# Autodesk Inventor assembly: Ensamble_Amortiguador
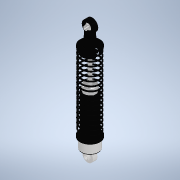
[picture p0: Inventor's stored thumbnail of the model, 180x180]
Saved by Autodesk Inventor 2020.2 (Build 242310000, 310)
## iProperties
Created: 2019-10-03
Part Number: Ensamble_Amortiguador
Document SubType Name: Assembly
Designer: axelj
Author: axelj
## Documents named in this file (11)
- C:\Users\axelj\OneDrive\Documentos\GitHub\autobot\robot_model\Ensamble_Amortiguador.iam
- C:\Users\axelj\OneDrive\Documentos\GitHub\autobot\robot_model\RCT-T005_Piston(Deposito_deAceite).ipt
- C:\Users\axelj\OneDrive\Documentos\GitHub\autobot\robot_model\RCT-T005_Embolo.ipt
- C:\Users\axelj\OneDrive\Documentos\GitHub\autobot\robot_model\RCT-T005_Elemento_externo.ipt
- C:\Users\axelj\OneDrive\Documentos\GitHub\autobot\robot_model\RCT-T005_Resorte.ipt
- C:\Users\axelj\OneDrive\Documentos\GitHub\autobot\robot_model\RCT-T005_Cubierta.ipt
- C:\Users\axelj\OneDrive\Documentos\GitHub\autobot\robot_model\RCT-T005_Conexion_superioript.ipt
- C:\Users\axelj\OneDrive\Documentos\GitHub\autobot\robot_model\RCT-T005_Pieza_Presion_resorte.ipt
- C:\Users\axelj\OneDrive\Documentos\GitHub\autobot\robot_model\RCT-T005_Conexion_inferior.ipt
- C:\Users\axelj\OneDrive\Documentos\GitHub\autobot\robot_model\RCT-H017_Bola_de_libertad_menor.ipt
- C:\Users\axelj\OneDrive\Documentos\GitHub\autobot\robot_model\RCT-H015_Bola_libertad_grande.ipt
## Components (10 placed, 10 different names)
1. RCT-T005_Piston(Deposito_deAceite):1 — Cilíndrica:1, Rígido:1, De rotación:1, De rotación:3
2. RCT-T005_Embolo:1 — Cilíndrica:1, De rotación:2
3. RCT-T005_Elemento_externo:1 — Rígido:1
4. RCT-T005_Resorte:1
5. RCT-T005_Cubierta:1 — De rotación:1
6. RCT-T005_Conexion_superioript:1 — De rotación:2, Rígido:2, De bola:1
7. RCT-T005_Pieza_Presion_resorte:1 — Rígido:2
8. RCT-T005_Conexion_inferior:1 — De rotación:3, De bola:2
9. RCT-H017_Bola_de_libertad_menor:1 — De bola:1
10. RCT-H015_Bola_libertad_grande:1 — De bola:2
## Relationships (8: RevoluteJoint 3, WeldJoint 2, BallJoint 2, CylindricalJoint 1)
- Cilíndrica:1 [CylindricalJoint]: RCT-T005_Piston(Deposito_deAceite):1 ↔ RCT-T005_Embolo:1
- Rígido:1 [WeldJoint]: RCT-T005_Piston(Deposito_deAceite):1 ↔ RCT-T005_Elemento_externo:1
- De rotación:1 [RevoluteJoint]: RCT-T005_Piston(Deposito_deAceite):1 ↔ RCT-T005_Cubierta:1
- De rotación:2 [RevoluteJoint]: RCT-T005_Embolo:1 ↔ RCT-T005_Conexion_superioript:1
- Rígido:2 [WeldJoint]: RCT-T005_Conexion_superioript:1 ↔ RCT-T005_Pieza_Presion_resorte:1
- De rotación:3 [RevoluteJoint] (0.001 mm): RCT-T005_Piston(Deposito_deAceite):1 ↔ RCT-T005_Conexion_inferior:1
- De bola:1 [BallJoint]: RCT-T005_Conexion_superioript:1 ↔ RCT-H017_Bola_de_libertad_menor:1
- De bola:2 [BallJoint]: RCT-T005_Conexion_inferior:1 ↔ RCT-H015_Bola_libertad_grande:1
